# Autodesk Inventor assembly: batteryMountingAssembly
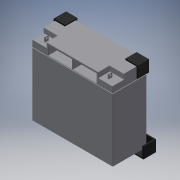
[picture p0: Inventor's stored thumbnail of the model, 180x180]
Saved by Autodesk Inventor 2017 (Build 210142000, 142)
## iProperties
Created: 2020-02-01
Part Number: batteryMountingAssembly
Document SubType Name: Assembly
Designer: S338674153
Author: S338674153
## Documents named in this file (4)
- \\ad.ocdsb.ca\studenthome\3\S338674153\FRC 2020\Modular Frame With 18in Brace\batteryMountingAssembly.iam
- \\ad.ocdsb.ca\studenthome\3\S338674153\FRC 2020\Modular Frame With 18in Brace\Battery.ipt
- \\ad.ocdsb.ca\studenthome\3\S338674153\FRC 2020\Modular Frame With 18in Brace\batteryCornerMount.ipt
- \\ad.ocdsb.ca\studenthome\3\S338674153\FRC 2020\Modular Frame With 18in Brace\batterymount.ipt
## Components (4 placed, 3 different names)
1. Battery:1 — Mate:1, Mate:2, Mate:3, Mate:4, Mate:5, Mate:6, Mate:7, Mate:8, Mate:9
2. batteryCornerMount:1 — Mate:4, Mate:5, Mate:6
3. batteryCornerMount:2 — Mate:1, Mate:2, Mate:3
4. batterymount:1 — Mate:7, Mate:8, Mate:9
## Relationships (9: Mate 9)
- Mate:1: Battery:1 ↔ batteryCornerMount:2
- Mate:2: Battery:1 ↔ batteryCornerMount:2
- Mate:3: Battery:1 ↔ batteryCornerMount:2
- Mate:4: Battery:1 ↔ batteryCornerMount:1
- Mate:5: Battery:1 ↔ batteryCornerMount:1
- Mate:6: Battery:1 ↔ batteryCornerMount:1
- Mate:7: Battery:1 ↔ batterymount:1
- Mate:8: Battery:1 ↔ batterymount:1
- Mate:9 (15.24 mm): Battery:1 ↔ batterymount:1
